# Autodesk Inventor assembly: Z Axis R
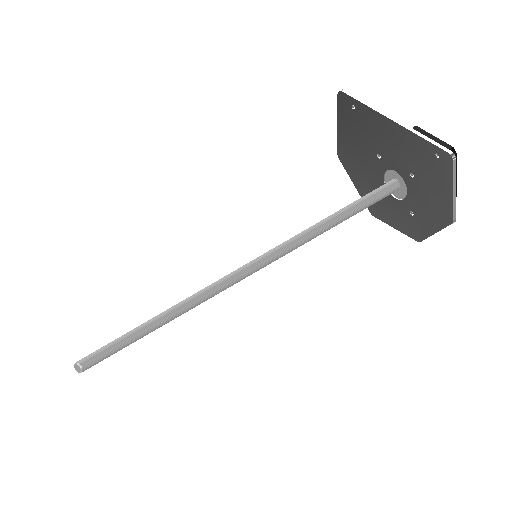
[picture p0: Inventor's stored thumbnail of the model, 512x512]
Saved by Autodesk Inventor 2023.2 (Build 272271000, 271)
## iProperties
Created: 2023-02-02
Part Number: Z Axis R
Document SubType Name: Assembly
Designer: remop
Author: remop
## Documents named in this file (3)
- C:\Users\remop\OneDrive\Documents\Inventor\3D Printers\LuEVO\Mk5_FullKinematic\Z Axis Rear.iam
- C:\Users\remop\OneDrive\Documents\Inventor\3D Printers\LuEVO\Mk5_FullKinematic\Z Axis Motor.ipt
- C:\Users\remop\OneDrive\Documents\Inventor\3D Printers\LuEVO\Mk5_FullKinematic\Z Axis Center Motor Mount.ipt
## Components (2 placed, 2 different names)
1. Z Axis Motor:1 — Flush:1
2. Z Axis Center Motor Mount:1 — Flush:1
## Relationships (1: Flush 1)
- Flush:1: Z Axis Motor:1 ↔ Z Axis Center Motor Mount:1
